# Autodesk Inventor assembly: wheelholder2
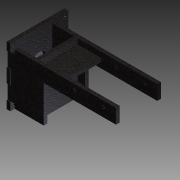
[picture p0: Inventor's stored thumbnail of the model, 180x180]
Saved by Autodesk Inventor 2011 (Build 150239000, 239)
## iProperties
Created: 2011-09-17
Part Number: wheelholder2
Document SubType Name: Assembly
Designer: Matthew
Author: Matthew
## Documents named in this file (6)
- C:\Users\Matthew\Documents\matthew_autocad\prlite\wheel\wheelholder2.iam
- C:\Users\Matthew\Documents\matthew_autocad\prlite\wheel\side 2.ipt
- C:\Users\Matthew\Documents\matthew_autocad\prlite\wheel\side 1.ipt
- C:\Users\Matthew\Documents\matthew_autocad\prlite\wheel\support 1.ipt
- C:\Users\Matthew\Documents\matthew_autocad\prlite\wheel\support 2.ipt
- C:\Users\Matthew\Documents\matthew_autocad\prlite\wheel\wheel top.ipt
## Components (5 placed, 5 different names)
1. support 1:1 — Flush:4, Mate:7, Mate:8, Flush:5, Mate:9
2. support 2:1 — Flush:4, Mate:7
3. wheel top:1 — Mate:10, Flush:6, Mate:11, Mate:12, Flush:7, Mate:13
4. side 1:1 — Mate:8, Flush:5, Mate:9, Mate:10, Flush:6, Mate:11
5. side 2:1 — Mate:12, Flush:7, Mate:13
## Relationships (11: Mate 7, Flush 4)
- Flush:4: support 1:1 ↔ support 2:1
- Mate:7: support 1:1 ↔ support 2:1
- Mate:8: support 1:1 ↔ side 1:1
- Flush:5: support 1:1 ↔ side 1:1
- Mate:9: support 1:1 ↔ side 1:1
- Mate:10: wheel top:1 ↔ side 1:1
- Flush:6: wheel top:1 ↔ side 1:1
- Mate:11: wheel top:1 ↔ side 1:1
- Mate:12: wheel top:1 ↔ side 2:1
- Flush:7: wheel top:1 ↔ side 2:1
- Mate:13: wheel top:1 ↔ side 2:1
